# Autodesk Inventor assembly: CenterShaft
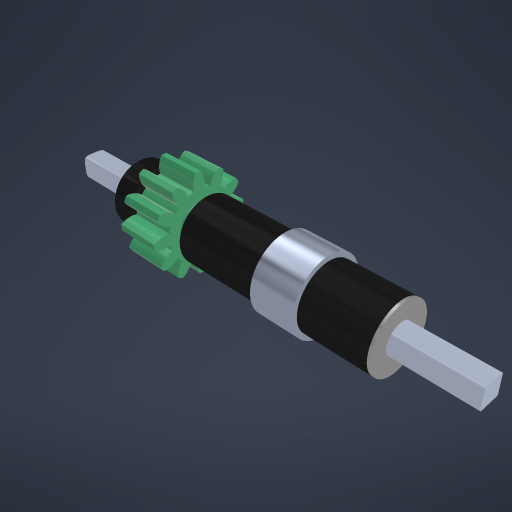
[picture p0: Inventor's stored thumbnail of the model, 512x512]
Saved by Autodesk Inventor 2023 (Build 270158000, 158)
## iProperties
Created: 2022-10-07
Part Number: CenterShaft
Document SubType Name: Assembly
Designer: alex
Author: alex
## Documents named in this file (11)
- C:\Users\alex\Documents\GitHub\4067X_spin_up_cad\Chassis\CenterShaft.iam
- C:\Users\alex\Documents\GitHub\4067X_spin_up_cad\Library\Motion\Spacers\Spacer Nylon .375 OD\NSpacer .375 OD x .125.ipt
- C:\Users\alex\Documents\GitHub\4067X_spin_up_cad\Library\Motion\Spacers\Spacer Nylon .375 OD.ipt
- C:\Users\alex\Documents\GitHub\4067X_spin_up_cad\Library\Motion\Gears\12T Gear.ipt
- C:\Users\alex\Documents\GitHub\4067X_spin_up_cad\Library\Motion\Spacers\Spacer Nylon .375 OD\NSpacer .375 OD x .500.ipt
- C:\Users\alex\Documents\GitHub\4067X_spin_up_cad\Library\Motion\Shaft Collar with Set Screw.ipt
- C:\Users\alex\Documents\GitHub\4067X_spin_up_cad\Library\Motion\Spacers\Spacer Nylon .375 OD\NSpacer .375 OD x .375.ipt
- C:\Users\alex\Documents\GitHub\4067X_spin_up_cad\Library\Motion\Spacers\Washer Steel\SWasher .375 OD x .015625.ipt
- C:\Users\alex\Documents\GitHub\4067X_spin_up_cad\Library\Motion\Spacers\Washer Steel.ipt
- C:\Users\alex\Documents\GitHub\4067X_spin_up_cad\Library\Motion\Shaft LS\Shaft LS 2.5 in.ipt
- C:\Users\alex\Documents\GitHub\4067X_spin_up_cad\Library\Motion\Shaft LS.ipt
## Components (7 placed, 7 different names)
1. NSpacer .375 OD x .125:1 — Insert:1, Flush:1
2. 12T Gear:1 — Insert:1, Mate:1, Mate:2, Insert:6
3. NSpacer .375 OD x .375:3 — Insert:5, Insert:8
4. SWasher .375 OD x .015625:1 — Insert:5
5. Shaft LS 2.5 in:1 — Mate:1, Mate:2, Flush:1
6. Shaft Collar with Set Screw:1 — Insert:7, Insert:8
7. NSpacer .375 OD x .500:4 — Insert:6, Insert:7
## Relationships (8: Insert 5, Mate 2, Flush 1)
- Insert:1: NSpacer .375 OD x .125:1 ↔ 12T Gear:1
- Insert:5: NSpacer .375 OD x .375:3 ↔ SWasher .375 OD x .015625:1
- Mate:1: 12T Gear:1 ↔ Shaft LS 2.5 in:1
- Mate:2: 12T Gear:1 ↔ Shaft LS 2.5 in:1
- Flush:1 (-10.9093 mm): NSpacer .375 OD x .125:1 ↔ Shaft LS 2.5 in:1
- Insert:6: 12T Gear:1 ↔ NSpacer .375 OD x .500:4
- Insert:7: Shaft Collar with Set Screw:1 ↔ NSpacer .375 OD x .500:4
- Insert:8: NSpacer .375 OD x .375:3 ↔ Shaft Collar with Set Screw:1
